# Autodesk Inventor assembly: Tank Tread Assembly
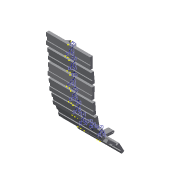
[picture p0: Inventor's stored thumbnail of the model, 180x180]
Saved by Autodesk Inventor 2015 (Build 190159000, 159)
## iProperties
Created: 2015-03-14
Part Number: Tank Tread Assembly
Document SubType Name: Assembly
Designer: james_000
Author: james_000
## Documents named in this file (3)
- C:\Users\james_000\Documents\Inventor\Test\Tank Tread Assembly.iam
- C:\Users\james_000\Documents\Inventor\Test\Tank Tread link A.ipt
- C:\Users\james_000\Documents\Inventor\Test\Tank Tread link B.ipt
## Components (16 placed, 2 different names)
1. Tank Tread link A:1 — Rotational:2, Rotational:3
2. Tank Tread link A:2 — Rotational:1
3. Tank Tread link B:1 — Rotational:1, Rotational:2
4. Tank Tread link B:2 — Rotational:3, Rotational:4
5. Tank Tread link A:3 — Rotational:4, Rotational:5
6. Tank Tread link B:3 — Rotational:5, Rotational:6
7. Tank Tread link B:4 — Rotational:7, Rotational:8
8. Tank Tread link B:5 — Rotational:9, Rotational:10
9. Tank Tread link B:6 — Rotational:11, Rotational:12
10. Tank Tread link B:7 — Rotational:13, Rotational:14
11. Tank Tread link B:8 — Rotational:15
12. Tank Tread link A:4 — Rotational:6, Rotational:7
13. Tank Tread link A:5 — Rotational:8, Rotational:9
14. Tank Tread link A:6 — Rotational:10, Rotational:11
15. Tank Tread link A:7 — Rotational:12, Rotational:13
16. Tank Tread link A:8 — Rotational:14, Rotational:15
## Relationships (15: RevoluteJoint 15)
- Rotational:1 [RevoluteJoint]: Tank Tread link A:2 ↔ Tank Tread link B:1
- Rotational:2 [RevoluteJoint]: Tank Tread link A:1 ↔ Tank Tread link B:1
- Rotational:3 [RevoluteJoint]: Tank Tread link A:1 ↔ Tank Tread link B:2
- Rotational:4 [RevoluteJoint]: Tank Tread link B:2 ↔ Tank Tread link A:3
- Rotational:5 [RevoluteJoint]: Tank Tread link A:3 ↔ Tank Tread link B:3
- Rotational:6 [RevoluteJoint]: Tank Tread link B:3 ↔ Tank Tread link A:4
- Rotational:7 [RevoluteJoint]: Tank Tread link B:4 ↔ Tank Tread link A:4
- Rotational:8 [RevoluteJoint]: Tank Tread link B:4 ↔ Tank Tread link A:5
- Rotational:9 [RevoluteJoint]: Tank Tread link B:5 ↔ Tank Tread link A:5
- Rotational:10 [RevoluteJoint]: Tank Tread link B:5 ↔ Tank Tread link A:6
- Rotational:11 [RevoluteJoint]: Tank Tread link B:6 ↔ Tank Tread link A:6
- Rotational:12 [RevoluteJoint]: Tank Tread link B:6 ↔ Tank Tread link A:7
- Rotational:13 [RevoluteJoint]: Tank Tread link B:7 ↔ Tank Tread link A:7
- Rotational:14 [RevoluteJoint]: Tank Tread link B:7 ↔ Tank Tread link A:8
- Rotational:15 [RevoluteJoint]: Tank Tread link B:8 ↔ Tank Tread link A:8
